# Autodesk Inventor assembly: Complete
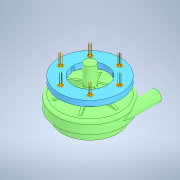
[picture p0: Inventor's stored thumbnail of the model, 180x180]
Saved by Autodesk Inventor 2022 (Build 260153000, 153)
## iProperties
Created: 2021-10-29
Part Number: Complete
Document SubType Name: Assembly
Designer: alber
Author: alber
## Documents named in this file (4)
- G:\My Drive\SPIN TEST Capstone\SpinTest_Capstone_Models\Complete.iam
- G:\My Drive\SPIN TEST Capstone\SpinTest_Capstone_Models\Pump_1.ipt
- G:\My Drive\SPIN TEST Capstone\SpinTest_Capstone_Models\Housing_1.ipt
- G:\My Drive\SPIN TEST Capstone\SpinTest_Capstone_Models\Sensor.ipt
## Components (8 placed, 3 different names)
1. Pump:1 — Cylindrical:1
2. Housing:1 — Cylindrical:1, Cylindrical:2, Cylindrical:3, Cylindrical:4, Cylindrical:5, Cylindrical:6, Cylindrical:7, Mate:1, Mate:2, Mate:3, Mate:4, Mate:5, Mate:6
3. Sensor:1 — Cylindrical:2, Mate:5
4. Sensor:2 — Cylindrical:4, Mate:4
5. Sensor:3 — Cylindrical:3, Mate:6
6. Sensor:4 — Cylindrical:5, Mate:2
7. Sensor:5 — Cylindrical:6, Mate:1
8. Sensor:6 — Cylindrical:7, Mate:3
## Relationships (13: CylindricalJoint 7, Mate 6)
- Cylindrical:1: Pump:1 ↔ Housing:1
- Cylindrical:2: Housing:1 ↔ Sensor:1
- Cylindrical:3: Housing:1 ↔ Sensor:3
- Cylindrical:4: Housing:1 ↔ Sensor:2
- Cylindrical:5: Housing:1 ↔ Sensor:4
- Cylindrical:6: Housing:1 ↔ Sensor:5
- Cylindrical:7: Housing:1 ↔ Sensor:6
- Mate:1: Housing:1 ↔ Sensor:5
- Mate:2: Housing:1 ↔ Sensor:4
- Mate:3: Housing:1 ↔ Sensor:6
- Mate:4: Housing:1 ↔ Sensor:2
- Mate:5: Housing:1 ↔ Sensor:1
- Mate:6: Housing:1 ↔ Sensor:3
